# Autodesk Inventor assembly: New vs Old Plate
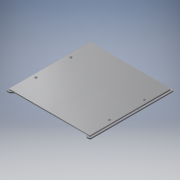
[picture p0: Inventor's stored thumbnail of the model, 180x180]
Saved by Autodesk Inventor 2017 (Build 210142000, 142)
## iProperties
Created: 2017-03-30
Part Number: New vs Old Plate
Document SubType Name: Assembly
Designer: gilef
Author: gilef
## Documents named in this file (3)
- C:\Users\gilef\Documents\Inventor\DiscoEasy200\New vs Old Plate.iam
- C:\Users\gilef\Documents\Inventor\DiscoEasy200\New Plate.ipt
- C:\Users\gilef\Documents\Inventor\DiscoEasy200\Stock Build Plate.ipt
## Components (2 placed, 2 different names)
1. New Plate:1 — Mate:1, Flush:1, Flush:2
2. Stock Build Plate:1 — Mate:1, Flush:1, Flush:2
## Relationships (3: Flush 2, Mate 1)
- Mate:1: New Plate:1 ↔ Stock Build Plate:1
- Flush:1 (4 mm): New Plate:1 ↔ Stock Build Plate:1
- Flush:2 (4 mm): New Plate:1 ↔ Stock Build Plate:1
